# Autodesk Inventor assembly: 2.75 Omni AS, No Insert_miirrored
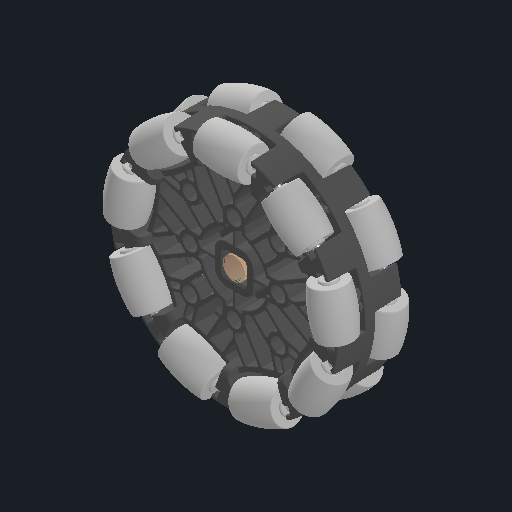
[picture p0: Inventor's stored thumbnail of the model, 512x512]
Saved by Autodesk Inventor 2025 (Build 290162000, 162)
## iProperties
Created: 2022-08-02
Part Number: 2.75 Omni AS, No Insert_miirrored
Document SubType Name: Assembly
Designer: Averey Ku
Author: ylu12
## Documents named in this file (2)
- D:\vex_robotics_high_stakes\hardware\cad\bots\high_stakes_v2\chassis\drivebay_mirrored\2.75 Omni AS, No Insert_miirrored.iam
- D:\vex_robotics_high_stakes\hardware\cad\bots\high_stakes_v2\chassis\drivebay_mirrored\2.75 Omni Antistatic_miirrored.ipt
## Components (1 placed, 1 different names)
1. 2.75 Omni Antistatic_miirrored:1 — Mate:8, Mate:7, Flush:4
## Relationships (3: Mate 2, Flush 1)
- Mate:8: 2.75 Omni Antistatic_miirrored:1
- Mate:7: 2.75 Omni Antistatic_miirrored:1
- Flush:4: 2.75 Omni Antistatic_miirrored:1
